# Autodesk Inventor assembly: visibleEnergy
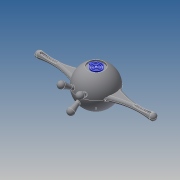
[picture p0: Inventor's stored thumbnail of the model, 180x180]
Saved by Autodesk Inventor 2017 (Build 210142000, 142)
## iProperties
Created: 2018-10-19
Part Number: visibleEnergy
Document SubType Name: Assembly
Designer: Gilles Mottiez
Author: Gilles Mottiez
## Documents named in this file (15)
- C:\Users\Gilles Mottiez\Documents\HES\I5_6\PGA\inventor\visibleEnergy.iam
- C:\Users\Gilles Mottiez\Documents\HES\I5_6\PGA\inventor\body_face.ipt
- C:\Users\Gilles Mottiez\Documents\HES\I5_6\PGA\inventor\ressort.ipt
- C:\Users\Gilles Mottiez\Documents\HES\I5_6\PGA\inventor\body_dos.ipt
- C:\Users\Gilles Mottiez\Documents\HES\I5_6\PGA\inventor\pieds.ipt
- C:\Users\Gilles Mottiez\Documents\HES\I5_6\PGA\inventor\plateforme_rpi_servo.iam
- C:\Users\Gilles Mottiez\Documents\HES\I5_6\PGA\inventor\arbre.ipt
- arbre.ipt
- C:\Users\Gilles Mottiez\Documents\HES\I5_6\PGA\inventor\palier_face.ipt
- palier_face.ipt
- C:\Users\Gilles Mottiez\Documents\HES\I5_6\PGA\inventor\axe.ipt
- axe.ipt
- C:\Users\Gilles Mottiez\Documents\HES\I5_6\PGA\inventor\bras_osc_dos.ipt
- bras_osc_dos.ipt
- C:\Users\Gilles Mottiez\Documents\HES\I5_6\PGA\inventor\bras_osc_front.ipt
## Components (14 placed, 9 different names)
1. body_face:1 — Placage:1, Placage:2, Logement:1, Logement:2, Logement:3, Logement:5, Placage:3, Placage:4, Logement:6
2. ressort:1 — Placage:1, Placage:2, Placage:5
3. body_dos:1 — Logement:1, Logement:2, Logement:4, Logement:8
4. pieds:1 — Logement:5
5. pieds:2 — Logement:4
6. pieds:3 — Logement:3
7. plateforme_rpi_servo:1 [sub-assembly] — Placage:3, Placage:4, Logement:9, Logement:10, Logement:11, Logement:12, Logement:13, Logement:15
8. arbre:1 — Logement:7, Placage:5
9. palier_face:1 — Logement:6, Logement:7
10. axe:1 — Logement:8
11. bras_osc_dos:1 — Logement:13, Logement:14
12. bras_osc_dos:2 — Logement:15, Logement:16
13. bras_osc_dos:3 — Logement:11, Logement:12, Logement:16
14. bras_osc_dos:4 — Logement:9, Logement:10, Logement:14
## Relationships (21: Insert 16, Mate 5)
- Placage:1 [Mate]: body_face:1 ↔ ressort:1
- Placage:2 [Mate]: body_face:1 ↔ ressort:1
- Logement:1 [Insert]: body_face:1 ↔ body_dos:1
- Logement:2 [Insert]: body_face:1 ↔ body_dos:1
- Logement:3 [Insert]: body_face:1 ↔ pieds:3
- Logement:4 [Insert]: body_dos:1 ↔ pieds:2
- Logement:5 [Insert]: body_face:1 ↔ pieds:1
- Placage:3 [Mate]: body_face:1 ↔ plateforme_rpi_servo:1
- Placage:4 [Mate]: body_face:1 ↔ plateforme_rpi_servo:1
- Logement:6 [Insert]: body_face:1 ↔ palier_face:1
- Logement:7 [Insert]: arbre:1 ↔ palier_face:1
- Placage:5 [Mate]: ressort:1 ↔ arbre:1
- Logement:8 [Insert]: body_dos:1 ↔ axe:1
- Logement:9 [Insert]: plateforme_rpi_servo:1 ↔ bras_osc_dos:4
- Logement:10 [Insert]: plateforme_rpi_servo:1 ↔ bras_osc_dos:4
- Logement:11 [Insert]: plateforme_rpi_servo:1 ↔ bras_osc_dos:3
- Logement:12 [Insert]: plateforme_rpi_servo:1 ↔ bras_osc_dos:3
- Logement:13 [Insert]: plateforme_rpi_servo:1 ↔ bras_osc_dos:1
- Logement:14 [Insert]: bras_osc_dos:1 ↔ bras_osc_dos:4
- Logement:15 [Insert]: plateforme_rpi_servo:1 ↔ bras_osc_dos:2
- Logement:16 [Insert]: bras_osc_dos:2 ↔ bras_osc_dos:3
